# Autodesk Inventor assembly: IntakeSlides5.0
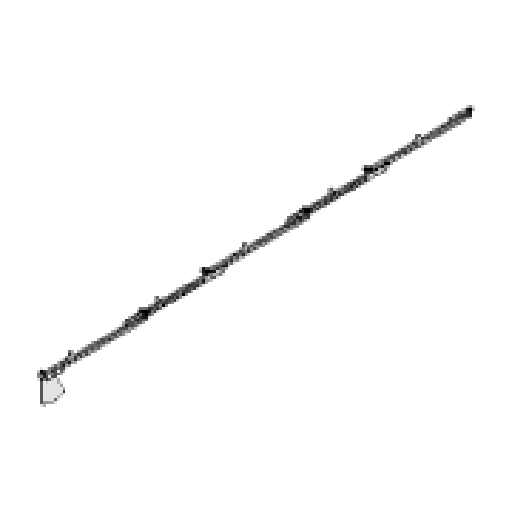
[picture p0: Inventor's stored thumbnail of the model, 512x512]
Saved by Autodesk Inventor 2023 (Build 270158000, 158)
## iProperties
Created: 2022-09-16
Part Number: IntakeSlides5.0
Document SubType Name: Assembly
Designer: deli
Author: deli
## Documents named in this file (13)
- C:\Users\deli\OneDrive - Eastside Preparatory School\FTC\8103-power-play\CAD\IntakeSlides5.0.iam
- C:\Users\deli\OneDrive - Eastside Preparatory School\FTC\8103-power-play\CAD\Carrige.ipt
- C:\Users\deli\OneDrive - Eastside Preparatory School\FTC\8103-power-play\CAD\FTC-parts\Mcmaster Carr\91294A126_Black-Oxide Alloy Steel Hex Drive Flat Head Screw.ipt
- C:\Users\deli\OneDrive - Eastside Preparatory School\FTC\8103-power-play\CAD\mgn9 350mm.ipt
- C:\Users\deli\OneDrive - Eastside Preparatory School\FTC\8103-power-play\CAD\Connector Plate350mm.ipt
- C:\Users\deli\OneDrive - Eastside Preparatory School\FTC\8103-power-play\CAD\mgn9SlideBearingHolder.ipt
- C:\Users\deli\OneDrive - Eastside Preparatory School\FTC\8103-power-play\CAD\Slides Bearings.iam
- C:\Users\deli\OneDrive - Eastside Preparatory School\FTC\8103-power-play\CAD\FTC-parts\M3\hex_socket_button_head_M3x14.ipt
- C:\Users\deli\OneDrive - Eastside Preparatory School\FTC\8103-power-play\CAD\intakeSlidesWheelHolder.ipt
- C:\Users\deli\OneDrive - Eastside Preparatory School\FTC\8103-power-play\CAD\Connector Plate350mm 2.ipt
- C:\Users\deli\OneDrive - Eastside Preparatory School\FTC\8103-power-play\CAD\FTC-parts\LongRobotics\3x12x4mm-bearing.ipt
- C:\Users\deli\OneDrive - Eastside Preparatory School\FTC\8103-power-play\CAD\M3 0.5mm Spacer.ipt
- C:\Users\deli\OneDrive - Eastside Preparatory School\FTC\8103-power-play\CAD\Cable Manegment.ipt
## Components (87 placed, 12 different names)
1. Carrige:3
2. Carrige:4 — Flush:21, Mate:29, Mate:30, Mate:31
3. 91294A126_Black-Oxide Alloy Steel Hex Drive Flat Head Screw:9 — Mate:36, Flush:25
4. 91294A126_Black-Oxide Alloy Steel Hex Drive Flat Head Screw:10 — Mate:34, Flush:28
5. 91294A126_Black-Oxide Alloy Steel Hex Drive Flat Head Screw:11 — Mate:38, Flush:23
6. 91294A126_Black-Oxide Alloy Steel Hex Drive Flat Head Screw:12 — Mate:39, Flush:24
7. 91294A126_Black-Oxide Alloy Steel Hex Drive Flat Head Screw:13 — Mate:32, Flush:29
8. 91294A126_Black-Oxide Alloy Steel Hex Drive Flat Head Screw:14 — Mate:35, Flush:27
9. 91294A126_Black-Oxide Alloy Steel Hex Drive Flat Head Screw:15 — Mate:33, Flush:26
10. 91294A126_Black-Oxide Alloy Steel Hex Drive Flat Head Screw:16 — Mate:37, Flush:22
11. mgn9 350mm:2 — Flush:21, Mate:94, Mate:98, Mate:233, Mate:250
12. Connector Plate350mm:1 — Mate:29, Mate:30, Mate:31, Mate:32, Mate:33, Mate:34, Mate:35, Mate:36, Mate:37, Mate:38, Mate:39, Flush:22, Flush:23, Flush:24, Flush:25, Flush:26, Flush:27, Flush:28, Flush:29, Mate:41, Mate:42, Mate:43, Mate:106, Mate:107, Angle:1, Mate:112, Mate:118, Angle:6, Flush:61, Mate:162, Mate:163, Mate:164, Mate:165, Mate:166, Mate:167, Mate:168, Mate:169, Flush:62, Flush:63, Flush:64, Flush:65, Flush:66, Flush:67, Flush:68
13. Carrige:5 — Mate:41, Mate:42
14. Carrige:6 — Mate:43, Mate:44, Mate:45, Flush:32
15. mgn9 350mm:3 — Mate:44, Mate:45, Flush:32, Mate:46, Mate:47, Mate:48, Mate:243, Mate:252
16. mgn9SlideBearingHolder:1 — Mate:46, Mate:47, Mate:48, Mate:80, Mate:198, Mate:212
17. Carrige:7 — Mate:147, Mate:151
18. Carrige:8 — Mate:152
19. 91294A126_Black-Oxide Alloy Steel Hex Drive Flat Head Screw:17 — Mate:155, Flush:60
20. 91294A126_Black-Oxide Alloy Steel Hex Drive Flat Head Screw:18 — Mate:158, Flush:55
21. 91294A126_Black-Oxide Alloy Steel Hex Drive Flat Head Screw:19 — Mate:154, Flush:59
22. 91294A126_Black-Oxide Alloy Steel Hex Drive Flat Head Screw:20 — Mate:156, Flush:58
23. 91294A126_Black-Oxide Alloy Steel Hex Drive Flat Head Screw:21 — Mate:149, Flush:53
24. 91294A126_Black-Oxide Alloy Steel Hex Drive Flat Head Screw:22 — Mate:157, Flush:56
25. 91294A126_Black-Oxide Alloy Steel Hex Drive Flat Head Screw:23 — Mate:153, Flush:57
26. 91294A126_Black-Oxide Alloy Steel Hex Drive Flat Head Screw:24 — Mate:150, Flush:54
27. mgn9 350mm:4 — Mate:80, Mate:236, Mate:237, Mate:238, Mate:251, Mate:253
28. Carrige:9 — Mate:159
29. Carrige:10 — Mate:160, Mate:161
30. mgn9 350mm:5 — Mate:142, Mate:143, Mate:144
31. mgn9SlideBearingHolder:3 — Mate:84, Mate:85, Mate:86, Mate:197, Mate:209
32. Carrige:11
33. Carrige:12
34. mgn9 350mm:6 — Mate:84, Mate:85, Mate:86, Mate:239, Mate:240, Mate:241
35. mgn9SlideBearingHolder:6 — Mate:95, Mate:96, Mate:97, Mate:98, Mate:199, Mate:214
36. Carrige:13
37. Carrige:14
38. mgn9 350mm:7 — Mate:94, Mate:95, Mate:96, Mate:97, Mate:234, Mate:235, Mate:242, Mate:244, Mate:245
39. Slides Bearings:3 [sub-assembly] — Mate:106, Mate:107, Angle:1, Mate:122, Mate:128
40. Slides Bearings:4 [sub-assembly] — Mate:112, Mate:118, Angle:6, Mate:136, Mate:137
41. Slides Bearings:8 [sub-assembly] — Mate:135, Mate:138, Mate:181, Angle:13
42. Slides Bearings:9 [sub-assembly] — Mate:126, Mate:127, Mate:180, Angle:12
43. hex_socket_button_head_M3x14:2 — Mate:122, Mate:128
44. hex_socket_button_head_M3x14:4 — Mate:126, Mate:127, Mate:178
45. hex_socket_button_head_M3x14:5 — Mate:136, Mate:137
46. hex_socket_button_head_M3x14:7 — Mate:135, Mate:138, Mate:179
47. hex_socket_button_head_M3x14:8 — Mate:202, Mate:204, Mate:209, Mate:210
48. hex_socket_button_head_M3x14:9 — Mate:201, Mate:208, Mate:211
49. hex_socket_button_head_M3x14:10 — Mate:200, Mate:207, Mate:213
50. intakeSlidesWheelHolder:1 — Mate:142, Mate:143, Mate:144, Mate:219, Mate:228
51. Connector Plate350mm 2:1 — Mate:147, Mate:149, Mate:150, Mate:151, Mate:152, Flush:53, Flush:54, Mate:153, Mate:154, Mate:155, Mate:156, Mate:157, Mate:158, Flush:55, Flush:56, Flush:57, Flush:58, Flush:59, Flush:60, Mate:159, Mate:160, Mate:161, Mate:170, Mate:171, Mate:172, Mate:173, Mate:174, Mate:175, Mate:176, Mate:177, Flush:69, Flush:70, Flush:71, Flush:72, Flush:73, Flush:74, Flush:75, Flush:76, Mate:178, Mate:179, Mate:180, Mate:181, Angle:12, Angle:13
52. 91294A126_Black-Oxide Alloy Steel Hex Drive Flat Head Screw:25 — Flush:61, Mate:162
53. 91294A126_Black-Oxide Alloy Steel Hex Drive Flat Head Screw:26 — Mate:167, Flush:63
54. 91294A126_Black-Oxide Alloy Steel Hex Drive Flat Head Screw:27 — Mate:163, Flush:68
55. 91294A126_Black-Oxide Alloy Steel Hex Drive Flat Head Screw:28 — Mate:165, Flush:64
56. 91294A126_Black-Oxide Alloy Steel Hex Drive Flat Head Screw:29 — Mate:168, Flush:65
57. 91294A126_Black-Oxide Alloy Steel Hex Drive Flat Head Screw:30 — Mate:166, Flush:67
58. 91294A126_Black-Oxide Alloy Steel Hex Drive Flat Head Screw:31 — Mate:169, Flush:62
59. 91294A126_Black-Oxide Alloy Steel Hex Drive Flat Head Screw:32 — Mate:164, Flush:66
60. 91294A126_Black-Oxide Alloy Steel Hex Drive Flat Head Screw:33 — Mate:170, Flush:71
61. 91294A126_Black-Oxide Alloy Steel Hex Drive Flat Head Screw:34 — Mate:171, Flush:69
62. 91294A126_Black-Oxide Alloy Steel Hex Drive Flat Head Screw:35 — Mate:177, Flush:75
63. 91294A126_Black-Oxide Alloy Steel Hex Drive Flat Head Screw:36 — Mate:176, Flush:74
64. 91294A126_Black-Oxide Alloy Steel Hex Drive Flat Head Screw:37 — Mate:175, Flush:76
65. 91294A126_Black-Oxide Alloy Steel Hex Drive Flat Head Screw:38 — Mate:172, Flush:72
66. 91294A126_Black-Oxide Alloy Steel Hex Drive Flat Head Screw:39 — Mate:173, Flush:70
67. 91294A126_Black-Oxide Alloy Steel Hex Drive Flat Head Screw:40 — Mate:174, Flush:73
68. 3x12x4mm-bearing:1 — Mate:205, Mate:208, Mate:211, Mate:212
69. 3x12x4mm-bearing:2 — Mate:206, Mate:207, Mate:213, Mate:214
70. 3x12x4mm-bearing:3 — Mate:203, Mate:204, Mate:210
71. M3 0.5mm Spacer:1 — Mate:197, Mate:202, Mate:203
72. M3 0.5mm Spacer:2 — Mate:199, Mate:200, Mate:206
73. M3 0.5mm Spacer:3 — Mate:198, Mate:201, Mate:205
74. hex_socket_button_head_M3x14:11 — Mate:217, Mate:228
75. 3x12x4mm-bearing:4 — Mate:218
76. M3 0.5mm Spacer:4 — Mate:217, Mate:218, Mate:219
77. hex_socket_button_head_M3x14:12 — Mate:249
78. 3x12x4mm-bearing:5
79. M3 0.5mm Spacer:5 — Mate:248
80. hex_socket_button_head_M3x14:13 — Mate:247
81. 3x12x4mm-bearing:6
82. M3 0.5mm Spacer:6 — Mate:246
83. Cable Manegment:1 — Mate:233, Mate:234, Mate:235
84. Cable Manegment:2 — Mate:236, Mate:237, Mate:238
85. Cable Manegment:3 — Mate:239, Mate:240, Mate:241
86. mgn9SlideBearingHolder:7 — Mate:243, Mate:248, Mate:249, Mate:251, Mate:252, Mate:253
87. mgn9SlideBearingHolder:8 — Mate:242, Mate:244, Mate:245, Mate:246, Mate:247, Mate:250
## Relationships (203: Mate 149, Flush 50, Angle 4)
- [Flush]: Carrige:3 ↔ Carrige:4
- [Flush]: Carrige:3 ↔ Carrige:4
- [Mate]: Carrige:3 ↔ Carrige:4
- [Mate]: Carrige:4 ↔ mgn9 350mm:2
- [Mate]: Carrige:4 ↔ mgn9 350mm:2
- Flush:21 (292.2 mm): Carrige:4 ↔ mgn9 350mm:2
- Mate:29: Carrige:4 ↔ Connector Plate350mm:1
- Mate:30: Carrige:4 ↔ Connector Plate350mm:1
- Mate:31: Carrige:4 ↔ Connector Plate350mm:1
- Mate:32: 91294A126_Black-Oxide Alloy Steel Hex Drive Flat Head Screw:13 ↔ Connector Plate350mm:1
- Mate:33: 91294A126_Black-Oxide Alloy Steel Hex Drive Flat Head Screw:15 ↔ Connector Plate350mm:1
- Mate:34: 91294A126_Black-Oxide Alloy Steel Hex Drive Flat Head Screw:10 ↔ Connector Plate350mm:1
- Mate:35: 91294A126_Black-Oxide Alloy Steel Hex Drive Flat Head Screw:14 ↔ Connector Plate350mm:1
- Mate:36: 91294A126_Black-Oxide Alloy Steel Hex Drive Flat Head Screw:9 ↔ Connector Plate350mm:1
- Mate:37: 91294A126_Black-Oxide Alloy Steel Hex Drive Flat Head Screw:16 ↔ Connector Plate350mm:1
- Mate:38: 91294A126_Black-Oxide Alloy Steel Hex Drive Flat Head Screw:11 ↔ Connector Plate350mm:1
- Mate:39: 91294A126_Black-Oxide Alloy Steel Hex Drive Flat Head Screw:12 ↔ Connector Plate350mm:1
- Flush:22: 91294A126_Black-Oxide Alloy Steel Hex Drive Flat Head Screw:16 ↔ Connector Plate350mm:1
- Flush:23: 91294A126_Black-Oxide Alloy Steel Hex Drive Flat Head Screw:11 ↔ Connector Plate350mm:1
- Flush:24: 91294A126_Black-Oxide Alloy Steel Hex Drive Flat Head Screw:12 ↔ Connector Plate350mm:1
- Flush:25: 91294A126_Black-Oxide Alloy Steel Hex Drive Flat Head Screw:9 ↔ Connector Plate350mm:1
- Flush:26: 91294A126_Black-Oxide Alloy Steel Hex Drive Flat Head Screw:15 ↔ Connector Plate350mm:1
- Flush:27: 91294A126_Black-Oxide Alloy Steel Hex Drive Flat Head Screw:14 ↔ Connector Plate350mm:1
- Flush:28: 91294A126_Black-Oxide Alloy Steel Hex Drive Flat Head Screw:10 ↔ Connector Plate350mm:1
- Flush:29: 91294A126_Black-Oxide Alloy Steel Hex Drive Flat Head Screw:13 ↔ Connector Plate350mm:1
- [Flush]: Carrige:5 ↔ Carrige:6
- [Flush]: Carrige:5 ↔ Carrige:6
- [Mate]: Carrige:5 ↔ Carrige:6
- Mate:41: Connector Plate350mm:1 ↔ Carrige:5
- Mate:42: Connector Plate350mm:1 ↔ Carrige:5
- Mate:43: Connector Plate350mm:1 ↔ Carrige:6
- Mate:44: Carrige:6 ↔ mgn9 350mm:3
- Mate:45: Carrige:6 ↔ mgn9 350mm:3
- Flush:32 (292.2 mm): Carrige:6 ↔ mgn9 350mm:3
- Mate:46: mgn9 350mm:3 ↔ mgn9SlideBearingHolder:1
- Mate:47: mgn9 350mm:3 ↔ mgn9SlideBearingHolder:1
- Mate:48: mgn9 350mm:3 ↔ mgn9SlideBearingHolder:1
- [Flush]: Carrige:7 ↔ Carrige:8
- [Flush]: Carrige:7 ↔ Carrige:8
- [Mate]: Carrige:7 ↔ Carrige:8
- [Mate]: Carrige:8 ↔ mgn9 350mm:4
- [Mate]: Carrige:8 ↔ mgn9 350mm:4
- [Flush] (292.2 mm): Carrige:8 ↔ mgn9 350mm:4
- [Flush]: Carrige:9 ↔ Carrige:10
- [Flush]: Carrige:9 ↔ Carrige:10
- [Mate]: Carrige:9 ↔ Carrige:10
- [Mate]: Carrige:10 ↔ mgn9 350mm:5
- [Mate]: Carrige:10 ↔ mgn9 350mm:5
- [Flush] (292.2 mm): Carrige:10 ↔ mgn9 350mm:5
- [Mate]: mgn9 350mm:5 ↔ mgn9SlideBearingHolder:3
- [Mate]: mgn9 350mm:5 ↔ mgn9SlideBearingHolder:3
- [Mate]: mgn9 350mm:5 ↔ mgn9SlideBearingHolder:3
- Mate:80: mgn9SlideBearingHolder:1 ↔ mgn9 350mm:4
- [Flush]: Carrige:11 ↔ Carrige:12
- [Flush]: Carrige:11 ↔ Carrige:12
- [Mate]: Carrige:11 ↔ Carrige:12
- [Mate]: Carrige:12 ↔ mgn9 350mm:6
- [Mate]: Carrige:12 ↔ mgn9 350mm:6
- [Flush] (292.2 mm): Carrige:12 ↔ mgn9 350mm:6
- Mate:84: mgn9SlideBearingHolder:3 ↔ mgn9 350mm:6
- Mate:85: mgn9SlideBearingHolder:3 ↔ mgn9 350mm:6
- Mate:86: mgn9SlideBearingHolder:3 ↔ mgn9 350mm:6
- [Flush]: Carrige:13 ↔ Carrige:14
- [Flush]: Carrige:13 ↔ Carrige:14
- [Mate]: Carrige:13 ↔ Carrige:14
- [Mate]: Carrige:14 ↔ mgn9 350mm:7
- [Mate]: Carrige:14 ↔ mgn9 350mm:7
- [Flush] (292.2 mm): Carrige:14 ↔ mgn9 350mm:7
- Mate:94: mgn9 350mm:2 ↔ mgn9 350mm:7
- Mate:95: mgn9SlideBearingHolder:6 ↔ mgn9 350mm:7
- Mate:96: mgn9SlideBearingHolder:6 ↔ mgn9 350mm:7
- Mate:97: mgn9SlideBearingHolder:6 ↔ mgn9 350mm:7
- Mate:98: mgn9 350mm:2 ↔ mgn9SlideBearingHolder:6
- Mate:106: Connector Plate350mm:1 ↔ Slides Bearings:3
- Mate:107: Connector Plate350mm:1 ↔ Slides Bearings:3
- Angle:1 (0 deg): Connector Plate350mm:1 ↔ Slides Bearings:3
- Mate:112: Connector Plate350mm:1 ↔ Slides Bearings:4
- Mate:118: Connector Plate350mm:1 ↔ Slides Bearings:4
- Angle:6 (0 deg): Connector Plate350mm:1 ↔ Slides Bearings:4
- Mate:122: Slides Bearings:3 ↔ hex_socket_button_head_M3x14:2
- Mate:126: Slides Bearings:9 ↔ hex_socket_button_head_M3x14:4
- Mate:127: Slides Bearings:9 ↔ hex_socket_button_head_M3x14:4
- Mate:128: Slides Bearings:3 ↔ hex_socket_button_head_M3x14:2
- Mate:135: Slides Bearings:8 ↔ hex_socket_button_head_M3x14:7
- Mate:136: Slides Bearings:4 ↔ hex_socket_button_head_M3x14:5
- Mate:137: Slides Bearings:4 ↔ hex_socket_button_head_M3x14:5
- Mate:138: Slides Bearings:8 ↔ hex_socket_button_head_M3x14:7
- Mate:142: mgn9 350mm:5 ↔ intakeSlidesWheelHolder:1
- Mate:143: mgn9 350mm:5 ↔ intakeSlidesWheelHolder:1
- Mate:144: mgn9 350mm:5 ↔ intakeSlidesWheelHolder:1
- Mate:147: Carrige:7 ↔ Connector Plate350mm 2:1
- Mate:149: 91294A126_Black-Oxide Alloy Steel Hex Drive Flat Head Screw:21 ↔ Connector Plate350mm 2:1
- Mate:150: 91294A126_Black-Oxide Alloy Steel Hex Drive Flat Head Screw:24 ↔ Connector Plate350mm 2:1
- Mate:151: Carrige:7 ↔ Connector Plate350mm 2:1
- Mate:152: Carrige:8 ↔ Connector Plate350mm 2:1
- Flush:53: 91294A126_Black-Oxide Alloy Steel Hex Drive Flat Head Screw:21 ↔ Connector Plate350mm 2:1
- Flush:54: 91294A126_Black-Oxide Alloy Steel Hex Drive Flat Head Screw:24 ↔ Connector Plate350mm 2:1
- Mate:153: 91294A126_Black-Oxide Alloy Steel Hex Drive Flat Head Screw:23 ↔ Connector Plate350mm 2:1
- Mate:154: 91294A126_Black-Oxide Alloy Steel Hex Drive Flat Head Screw:19 ↔ Connector Plate350mm 2:1
- Mate:155: 91294A126_Black-Oxide Alloy Steel Hex Drive Flat Head Screw:17 ↔ Connector Plate350mm 2:1
- Mate:156: 91294A126_Black-Oxide Alloy Steel Hex Drive Flat Head Screw:20 ↔ Connector Plate350mm 2:1
- Mate:157: 91294A126_Black-Oxide Alloy Steel Hex Drive Flat Head Screw:22 ↔ Connector Plate350mm 2:1
- Mate:158: 91294A126_Black-Oxide Alloy Steel Hex Drive Flat Head Screw:18 ↔ Connector Plate350mm 2:1
- Flush:55: 91294A126_Black-Oxide Alloy Steel Hex Drive Flat Head Screw:18 ↔ Connector Plate350mm 2:1
- Flush:56: 91294A126_Black-Oxide Alloy Steel Hex Drive Flat Head Screw:22 ↔ Connector Plate350mm 2:1
- Flush:57: 91294A126_Black-Oxide Alloy Steel Hex Drive Flat Head Screw:23 ↔ Connector Plate350mm 2:1
- Flush:58: 91294A126_Black-Oxide Alloy Steel Hex Drive Flat Head Screw:20 ↔ Connector Plate350mm 2:1
- Flush:59: 91294A126_Black-Oxide Alloy Steel Hex Drive Flat Head Screw:19 ↔ Connector Plate350mm 2:1
- Flush:60: 91294A126_Black-Oxide Alloy Steel Hex Drive Flat Head Screw:17 ↔ Connector Plate350mm 2:1
- Mate:159: Carrige:9 ↔ Connector Plate350mm 2:1
- Mate:160: Carrige:10 ↔ Connector Plate350mm 2:1
- Mate:161: Carrige:10 ↔ Connector Plate350mm 2:1
- Flush:61: Connector Plate350mm:1 ↔ 91294A126_Black-Oxide Alloy Steel Hex Drive Flat Head Screw:25
- Mate:162: Connector Plate350mm:1 ↔ 91294A126_Black-Oxide Alloy Steel Hex Drive Flat Head Screw:25
- Mate:163: Connector Plate350mm:1 ↔ 91294A126_Black-Oxide Alloy Steel Hex Drive Flat Head Screw:27
- Mate:164: Connector Plate350mm:1 ↔ 91294A126_Black-Oxide Alloy Steel Hex Drive Flat Head Screw:32
- Mate:165: Connector Plate350mm:1 ↔ 91294A126_Black-Oxide Alloy Steel Hex Drive Flat Head Screw:28
- Mate:166: Connector Plate350mm:1 ↔ 91294A126_Black-Oxide Alloy Steel Hex Drive Flat Head Screw:30
- Mate:167: Connector Plate350mm:1 ↔ 91294A126_Black-Oxide Alloy Steel Hex Drive Flat Head Screw:26
- Mate:168: Connector Plate350mm:1 ↔ 91294A126_Black-Oxide Alloy Steel Hex Drive Flat Head Screw:29
- Mate:169: Connector Plate350mm:1 ↔ 91294A126_Black-Oxide Alloy Steel Hex Drive Flat Head Screw:31
- Flush:62: Connector Plate350mm:1 ↔ 91294A126_Black-Oxide Alloy Steel Hex Drive Flat Head Screw:31
- Flush:63: Connector Plate350mm:1 ↔ 91294A126_Black-Oxide Alloy Steel Hex Drive Flat Head Screw:26
- Flush:64: Connector Plate350mm:1 ↔ 91294A126_Black-Oxide Alloy Steel Hex Drive Flat Head Screw:28
- Flush:65: Connector Plate350mm:1 ↔ 91294A126_Black-Oxide Alloy Steel Hex Drive Flat Head Screw:29
- Flush:66: Connector Plate350mm:1 ↔ 91294A126_Black-Oxide Alloy Steel Hex Drive Flat Head Screw:32
- Flush:67: Connector Plate350mm:1 ↔ 91294A126_Black-Oxide Alloy Steel Hex Drive Flat Head Screw:30
- Flush:68: Connector Plate350mm:1 ↔ 91294A126_Black-Oxide Alloy Steel Hex Drive Flat Head Screw:27
- Mate:170: Connector Plate350mm 2:1 ↔ 91294A126_Black-Oxide Alloy Steel Hex Drive Flat Head Screw:33
- Mate:171: Connector Plate350mm 2:1 ↔ 91294A126_Black-Oxide Alloy Steel Hex Drive Flat Head Screw:34
- Mate:172: Connector Plate350mm 2:1 ↔ 91294A126_Black-Oxide Alloy Steel Hex Drive Flat Head Screw:38
- Mate:173: Connector Plate350mm 2:1 ↔ 91294A126_Black-Oxide Alloy Steel Hex Drive Flat Head Screw:39
- Mate:174: Connector Plate350mm 2:1 ↔ 91294A126_Black-Oxide Alloy Steel Hex Drive Flat Head Screw:40
- Mate:175: Connector Plate350mm 2:1 ↔ 91294A126_Black-Oxide Alloy Steel Hex Drive Flat Head Screw:37
- Mate:176: Connector Plate350mm 2:1 ↔ 91294A126_Black-Oxide Alloy Steel Hex Drive Flat Head Screw:36
- Mate:177: Connector Plate350mm 2:1 ↔ 91294A126_Black-Oxide Alloy Steel Hex Drive Flat Head Screw:35
- Flush:69: Connector Plate350mm 2:1 ↔ 91294A126_Black-Oxide Alloy Steel Hex Drive Flat Head Screw:34
- Flush:70: Connector Plate350mm 2:1 ↔ 91294A126_Black-Oxide Alloy Steel Hex Drive Flat Head Screw:39
- Flush:71: Connector Plate350mm 2:1 ↔ 91294A126_Black-Oxide Alloy Steel Hex Drive Flat Head Screw:33
- Flush:72: Connector Plate350mm 2:1 ↔ 91294A126_Black-Oxide Alloy Steel Hex Drive Flat Head Screw:38
- Flush:73: Connector Plate350mm 2:1 ↔ 91294A126_Black-Oxide Alloy Steel Hex Drive Flat Head Screw:40
- Flush:74: Connector Plate350mm 2:1 ↔ 91294A126_Black-Oxide Alloy Steel Hex Drive Flat Head Screw:36
- Flush:75: Connector Plate350mm 2:1 ↔ 91294A126_Black-Oxide Alloy Steel Hex Drive Flat Head Screw:35
- Flush:76: Connector Plate350mm 2:1 ↔ 91294A126_Black-Oxide Alloy Steel Hex Drive Flat Head Screw:37
- Mate:178: hex_socket_button_head_M3x14:4 ↔ Connector Plate350mm 2:1
- Mate:179: hex_socket_button_head_M3x14:7 ↔ Connector Plate350mm 2:1
- Mate:180: Slides Bearings:9 ↔ Connector Plate350mm 2:1
- Mate:181: Slides Bearings:8 ↔ Connector Plate350mm 2:1
- Angle:12 (0 deg): Slides Bearings:9 ↔ Connector Plate350mm 2:1
- Angle:13 (0 deg): Slides Bearings:8 ↔ Connector Plate350mm 2:1
- Mate:197: mgn9SlideBearingHolder:3 ↔ M3 0.5mm Spacer:1
- Mate:198: mgn9SlideBearingHolder:1 ↔ M3 0.5mm Spacer:3
- Mate:199: mgn9SlideBearingHolder:6 ↔ M3 0.5mm Spacer:2
- Mate:200: hex_socket_button_head_M3x14:10 ↔ M3 0.5mm Spacer:2
- Mate:201: hex_socket_button_head_M3x14:9 ↔ M3 0.5mm Spacer:3
- Mate:202: hex_socket_button_head_M3x14:8 ↔ M3 0.5mm Spacer:1
- Mate:203: 3x12x4mm-bearing:3 ↔ M3 0.5mm Spacer:1
- Mate:204: hex_socket_button_head_M3x14:8 ↔ 3x12x4mm-bearing:3
- Mate:205: 3x12x4mm-bearing:1 ↔ M3 0.5mm Spacer:3
- Mate:206: 3x12x4mm-bearing:2 ↔ M3 0.5mm Spacer:2
- Mate:207: hex_socket_button_head_M3x14:10 ↔ 3x12x4mm-bearing:2
- Mate:208: hex_socket_button_head_M3x14:9 ↔ 3x12x4mm-bearing:1
- Mate:209: mgn9SlideBearingHolder:3 ↔ hex_socket_button_head_M3x14:8
- Mate:210: hex_socket_button_head_M3x14:8 ↔ 3x12x4mm-bearing:3
- Mate:211: hex_socket_button_head_M3x14:9 ↔ 3x12x4mm-bearing:1
- Mate:212: mgn9SlideBearingHolder:1 ↔ 3x12x4mm-bearing:1
- Mate:213: hex_socket_button_head_M3x14:10 ↔ 3x12x4mm-bearing:2
- Mate:214: mgn9SlideBearingHolder:6 ↔ 3x12x4mm-bearing:2
- [Mate]: hex_socket_button_head_M3x14:11 ↔ 3x12x4mm-bearing:4
- [Mate]: hex_socket_button_head_M3x14:11 ↔ 3x12x4mm-bearing:4
- Mate:217: hex_socket_button_head_M3x14:11 ↔ M3 0.5mm Spacer:4
- Mate:218: 3x12x4mm-bearing:4 ↔ M3 0.5mm Spacer:4
- Mate:219: intakeSlidesWheelHolder:1 ↔ M3 0.5mm Spacer:4
- [Mate]: hex_socket_button_head_M3x14:12 ↔ 3x12x4mm-bearing:5
- [Mate]: hex_socket_button_head_M3x14:12 ↔ 3x12x4mm-bearing:5
- [Mate]: hex_socket_button_head_M3x14:12 ↔ M3 0.5mm Spacer:5
- [Mate]: 3x12x4mm-bearing:5 ↔ M3 0.5mm Spacer:5
- [Mate]: hex_socket_button_head_M3x14:13 ↔ 3x12x4mm-bearing:6
- [Mate]: hex_socket_button_head_M3x14:13 ↔ 3x12x4mm-bearing:6
- [Mate]: hex_socket_button_head_M3x14:13 ↔ M3 0.5mm Spacer:6
- [Mate]: 3x12x4mm-bearing:6 ↔ M3 0.5mm Spacer:6
- Mate:228: intakeSlidesWheelHolder:1 ↔ hex_socket_button_head_M3x14:11
- Mate:233: mgn9 350mm:2 ↔ Cable Manegment:1
- Mate:234: mgn9 350mm:7 ↔ Cable Manegment:1
- Mate:235: mgn9 350mm:7 ↔ Cable Manegment:1
- Mate:236: mgn9 350mm:4 ↔ Cable Manegment:2
- Mate:237: mgn9 350mm:4 ↔ Cable Manegment:2
- Mate:238: mgn9 350mm:4 ↔ Cable Manegment:2
- Mate:239: mgn9 350mm:6 ↔ Cable Manegment:3
- Mate:240: mgn9 350mm:6 ↔ Cable Manegment:3
- Mate:241: mgn9 350mm:6 ↔ Cable Manegment:3
- Mate:242: mgn9 350mm:7 ↔ mgn9SlideBearingHolder:8
- Mate:243: mgn9 350mm:3 ↔ mgn9SlideBearingHolder:7
- Mate:244: mgn9 350mm:7 ↔ mgn9SlideBearingHolder:8
- Mate:245: mgn9 350mm:7 ↔ mgn9SlideBearingHolder:8
- Mate:246: M3 0.5mm Spacer:6 ↔ mgn9SlideBearingHolder:8
- Mate:247: hex_socket_button_head_M3x14:13 ↔ mgn9SlideBearingHolder:8
- Mate:248: M3 0.5mm Spacer:5 ↔ mgn9SlideBearingHolder:7
- Mate:249: hex_socket_button_head_M3x14:12 ↔ mgn9SlideBearingHolder:7
- Mate:250: mgn9 350mm:2 ↔ mgn9SlideBearingHolder:8
- Mate:251: mgn9 350mm:4 ↔ mgn9SlideBearingHolder:7
- Mate:252: mgn9 350mm:3 ↔ mgn9SlideBearingHolder:7
- Mate:253: mgn9 350mm:4 ↔ mgn9SlideBearingHolder:7
## Named parameters: stroke = 292.2 mm, d170_d117 = 0 mm, d171_d118 = 0 mm, d172_d119 = 0 mm, d192_d148 = 0 mm, d542_d170_d117 = 0 mm, d543_d171_d118 = 0 mm, d544_d172_d119 = 0 mm, d565_d149 = 0 mm, d566_d170_d117 = 0 mm, d567_d171_d118 = 0 mm, d568_d172_d119 = 0 mm, d569_d192_d148 = 0 mm, d570_d330 = 292.2 mm, d585_d542_d170_d117 = 0 mm, d586_d543_d171_d118 = 0 mm, d587_d544_d172_d119 = 0 mm, d591_d548 = 0 mm, d592_d549 = 0 mm, d593_d550 = 292.2 mm, d594_d551 = 0 mm, d595_d552 = 0 mm, d596_d553 = 0 mm, d603_d565_d149 = 0 mm, d604_d566_d170_d117 = 0 mm, d605_d567_d171_d118 = 0 mm, d606_d568_d172_d119 = 0 mm, d607_d569_d192_d148 = 0 mm, d608_d570_d330 = 292.2 mm, d613_d603_d565_d149 = 0 mm, d614_d604_d566_d170_d117 = 0 mm, d615_d605_d567_d171_d118 = 0 mm, d616_d606_d568_d172_d119 = 0 mm, d617_d607_d569_d192_d148 = 0 mm, d618_d608_d570_d330 = 292.2 mm, d785_d774 = 0 mm, d786_d780 = 0 mm, d790_d785_d774 = 0 mm, d791_d786_d780 = 0 mm, d792_d787 = 0 mm, d793_d788 = 0 mm, d794_d785_d774 = 0 mm, d795_d786_d780 = 0 mm, d796_d787 = 0 mm, d797_d788 = 0 mm
